# Autodesk Inventor assembly: Assem220Kicker
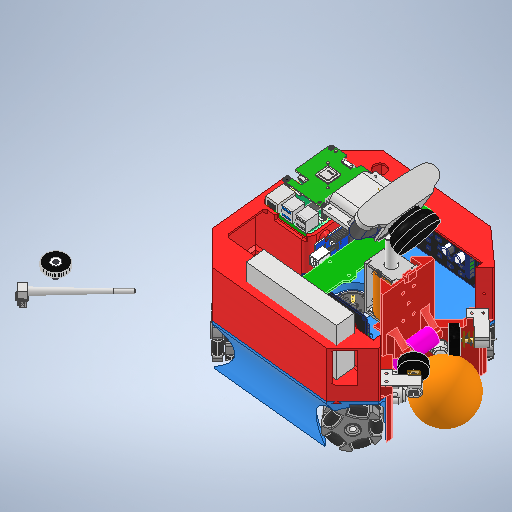
[picture p0: Inventor's stored thumbnail of the model, 512x512]
Saved by Autodesk Inventor 2025.1 (Build 291241000, 241)
## iProperties
Created: 2025-05-09
Part Number: Assem220Kicker
Document SubType Name: Assembly
Designer: User
Author: User
## Documents named in this file (23)
- D:\One Drive\OneDrive - Politeknik Sultan Salahuddin Abdul Aziz Shah\Documents\Inventor\RobosotPSA\Assem220Kicker.iam
- D:\One Drive\OneDrive - Politeknik Sultan Salahuddin Abdul Aziz Shah\Documents\Inventor\RobosotPSA\WheelMotor.iam
- D:\One Drive\OneDrive - Politeknik Sultan Salahuddin Abdul Aziz Shah\Documents\Inventor\RobosotPSA\MainBaseKicker.ipt
- D:\One Drive\OneDrive - Politeknik Sultan Salahuddin Abdul Aziz Shah\Documents\Inventor\RobosotPSA\Solenoid - 35mm Push-Pull\Solenoid - 35mm Push-Pull\Solenoid - 35mm Push-Pull.ipt
- D:\One Drive\OneDrive - Politeknik Sultan Salahuddin Abdul Aziz Shah\Documents\Inventor\RobosotPSA\Capacitor1.ipt
- D:\One Drive\OneDrive - Politeknik Sultan Salahuddin Abdul Aziz Shah\Documents\Inventor\RobosotPSA\CapCharger.ipt
- D:\One Drive\OneDrive - Politeknik Sultan Salahuddin Abdul Aziz Shah\Documents\Inventor\RobosotPSA\Kicker.ipt
- D:\One Drive\OneDrive - Politeknik Sultan Salahuddin Abdul Aziz Shah\Documents\Inventor\RobosotPSA\MainBox.ipt
- D:\One Drive\OneDrive - Politeknik Sultan Salahuddin Abdul Aziz Shah\Documents\Inventor\RobosotPSA\RPIassem.iam
- D:\One Drive\OneDrive - Politeknik Sultan Salahuddin Abdul Aziz Shah\Documents\Inventor\RobosotPSA\Motor Driver\Motor Driver\Motor Driver.ipt
- D:\One Drive\OneDrive - Politeknik Sultan Salahuddin Abdul Aziz Shah\Documents\Inventor\RobosotPSA\Arduino_Mega\Arduino_Mega\Arduino_Mega.ipt
- D:\One Drive\OneDrive - Politeknik Sultan Salahuddin Abdul Aziz Shah\Documents\Inventor\RobosotPSA\LiPo3000mAH.ipt
- D:\One Drive\OneDrive - Politeknik Sultan Salahuddin Abdul Aziz Shah\Documents\Inventor\RobosotPSA\TheBall70mm.ipt
- D:\One Drive\OneDrive - Politeknik Sultan Salahuddin Abdul Aziz Shah\Documents\Inventor\RobosotPSA\caster_wheel_15mm\caster_wheel_15mm\caster_wheel_15mm.ipt
- D:\One Drive\OneDrive - Politeknik Sultan Salahuddin Abdul Aziz Shah\Documents\Inventor\RobosotPSA\SwingKicker.ipt
- D:\One Drive\OneDrive - Politeknik Sultan Salahuddin Abdul Aziz Shah\Documents\Inventor\RobosotPSA\N20 Mini Micro Metall Gear Motor DC 3-6-12V v1\N20 Mini Micro Metall Gear Motor DC 3-6-12V v1\N20 Mini Micro Me.ipt
- D:\One Drive\OneDrive - Politeknik Sultan Salahuddin Abdul Aziz Shah\Documents\Inventor\RobosotPSA\DribbleWheel.ipt
- D:\One Drive\OneDrive - Politeknik Sultan Salahuddin Abdul Aziz Shah\Documents\Inventor\RobosotPSA\leftWheeler.ipt
- D:\One Drive\OneDrive - Politeknik Sultan Salahuddin Abdul Aziz Shah\Documents\Inventor\RobosotPSA\rightWheeler.ipt
- D:\One Drive\OneDrive - Politeknik Sultan Salahuddin Abdul Aziz Shah\Documents\Inventor\RobosotPSA\Logitech_C920.iam
- D:\One Drive\OneDrive - Politeknik Sultan Salahuddin Abdul Aziz Shah\Documents\Inventor\RobosotPSA\CameraPlate.ipt
- D:\One Drive\OneDrive - Politeknik Sultan Salahuddin Abdul Aziz Shah\Documents\Inventor\RobosotPSA\rpiCameraMAssembly\RJ45 Port Cap_Slim.ipt
- D:\One Drive\OneDrive - Politeknik Sultan Salahuddin Abdul Aziz Shah\Documents\Inventor\RobosotPSA\Kamera_Schraube_Tripod\Kamera_Schraube_Tripod\Kamera_Schraube_Tripod.ipt
## Components (32 placed, 22 different names)
1. MainBaseKicker:1 — Flush:1, Flush:2, Mate:2, Mate:3, Mate:4, Flush:3, Flush:4, Mate:5, Mate:12, Flush:5
2. Solenoid - 35mm Push-Pull:1 — Flush:2, Mate:2
3. Capacitor1:1
4. Capacitor1:2
5. CapCharger:1 — Mate:3, Mate:4
6. Kicker:1 — Flush:3, Mate:13, Mate:14, Mate:15, Mate:16, Mate:17, Mate:18, Mate:22, Mate:23
7. MainBox:1 — Flush:4, Flush:7
8. RPIassem:1 [sub-assembly] — Mate:5, Mate:9
9. Motor Driver:1
10. Motor Driver:2
11. Arduino_Mega:1 — Mate:9
12. LiPo3000mAH:1 — Mate:12, Flush:5
13. TheBall70mm:1
14. caster_wheel_15mm:1 — Mate:13
15. caster_wheel_15mm:2 — Mate:14
16. caster_wheel_15mm:3 — Mate:15
17. caster_wheel_15mm:4 — Mate:16
18. SwingKicker:1 — Mate:17, Mate:18
19. N20 Mini Micro Me:1 — Mate:20, Mate:22, Mate:24, Mate:25, Mate:26
20. DribbleWheel:1 — Mate:20
21. N20 Mini Micro Me:2 — Mate:19, Mate:21, Mate:23, Flush:6
22. DribbleWheel:2 — Mate:19, Mate:21
23. leftWheeler:1 — Flush:6
24. rightWheeler:1 — Mate:24, Mate:25, Mate:26
25. Logitech_C920:1 [sub-assembly]
26. CameraPlate:1 — Flush:7
27. RJ45 Port Cap_Slim:1
28. Kamera_Schraube_Tripod:1
29. WheelMotor:1 [sub-assembly] — Flush:1
30. WheelMotor:2 [sub-assembly]
31. WheelMotor:3 [sub-assembly]
32. WheelMotor:4 [sub-assembly]
## Component patterns: (4 elements, first: WheelMotor:1)
## Relationships (27: Mate 20, Flush 7)
- Flush:1: MainBaseKicker:1 ↔ WheelMotor:1
- Flush:2 (40 mm): MainBaseKicker:1 ↔ Solenoid - 35mm Push-Pull:1
- Mate:2 (20 mm): MainBaseKicker:1 ↔ Solenoid - 35mm Push-Pull:1
- Mate:3 (-4 mm): MainBaseKicker:1 ↔ CapCharger:1
- Mate:4: MainBaseKicker:1 ↔ CapCharger:1
- Flush:3: MainBaseKicker:1 ↔ Kicker:1
- Flush:4: MainBaseKicker:1 ↔ MainBox:1
- Mate:5 (7 mm): MainBaseKicker:1 ↔ RPIassem:1
- Mate:9 (10 mm): RPIassem:1 ↔ Arduino_Mega:1
- Mate:12 (25 mm): MainBaseKicker:1 ↔ LiPo3000mAH:1
- Flush:5 (10 mm): MainBaseKicker:1 ↔ LiPo3000mAH:1
- Mate:13: Kicker:1 ↔ caster_wheel_15mm:1
- Mate:14: Kicker:1 ↔ caster_wheel_15mm:2
- Mate:15: Kicker:1 ↔ caster_wheel_15mm:3
- Mate:16: Kicker:1 ↔ caster_wheel_15mm:4
- Mate:17 (1 mm): Kicker:1 ↔ SwingKicker:1
- Mate:18: Kicker:1 ↔ SwingKicker:1
- Mate:19: N20 Mini Micro Me:2 ↔ DribbleWheel:2
- Mate:20 (-15 mm): N20 Mini Micro Me:1 ↔ DribbleWheel:1
- Mate:21 (-15 mm): N20 Mini Micro Me:2 ↔ DribbleWheel:2
- Mate:22: Kicker:1 ↔ N20 Mini Micro Me:1
- Mate:23: Kicker:1 ↔ N20 Mini Micro Me:2
- Flush:6: N20 Mini Micro Me:2 ↔ leftWheeler:1
- Mate:24 (0.5 mm): N20 Mini Micro Me:1 ↔ rightWheeler:1
- Mate:25 (0.5 mm): N20 Mini Micro Me:1 ↔ rightWheeler:1
- Mate:26: N20 Mini Micro Me:1 ↔ rightWheeler:1
- Flush:7: MainBox:1 ↔ CameraPlate:1
